# Autodesk Inventor assembly: Arcade
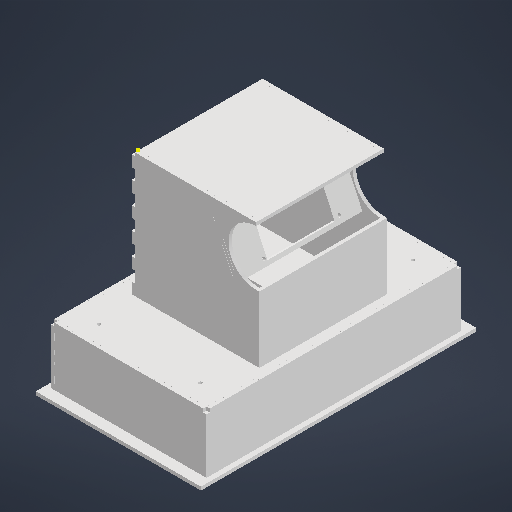
[picture p0: Inventor's stored thumbnail of the model, 512x512]
Saved by Autodesk Inventor 2026 (Build 300175000, 175)
## iProperties
Created: 2026-04-21
Part Number: Arcade
Document SubType Name: Assembly
Designer: juana
Author: juana
## Documents named in this file (9)
- C:\Users\juana\OneDrive\Documentos\GitHub\Digital_2\ModuloSTM32\ProyectoVideoJuegoF401RE\Arcade\Arcade.iam
- C:\Users\juana\OneDrive\Documentos\GitHub\Digital_2\ModuloSTM32\ProyectoVideoJuegoF401RE\Arcade\base.ipt
- C:\Users\juana\OneDrive\Documentos\GitHub\Digital_2\ModuloSTM32\ProyectoVideoJuegoF401RE\Arcade\AnchoBase.ipt
- C:\Users\juana\OneDrive\Documentos\GitHub\Digital_2\ModuloSTM32\ProyectoVideoJuegoF401RE\Arcade\paredBase.ipt
- C:\Users\juana\OneDrive\Documentos\GitHub\Digital_2\ModuloSTM32\ProyectoVideoJuegoF401RE\Arcade\ParedPantalla.ipt
- C:\Users\juana\OneDrive\Documentos\GitHub\Digital_2\ModuloSTM32\ProyectoVideoJuegoF401RE\Arcade\Techo.ipt
- C:\Users\juana\OneDrive\Documentos\GitHub\Digital_2\ModuloSTM32\ProyectoVideoJuegoF401RE\Arcade\portada.ipt
- C:\Users\juana\OneDrive\Documentos\GitHub\Digital_2\ModuloSTM32\ProyectoVideoJuegoF401RE\Arcade\pantallaSoport.ipt
- C:\Users\juana\OneDrive\Documentos\GitHub\Digital_2\ModuloSTM32\ProyectoVideoJuegoF401RE\Arcade\Techopantalla.ipt
## Components (11 placed, 8 different names)
1. base:1 — Mate:1, Mate:2, Flush:1, Mate:3, Mate:6, Flush:2, Mate:7, Mate:8
2. Techo:1 — Mate:9, Flush:3, Mate:10, Mate:11, Mate:12, Mate:13, Mate:14
3. portada:1 — Flush:4, Mate:14, Mate:15
4. pantallaSoport:1 — Flush:5, Mate:16, Mate:17
5. Techopantalla:1 — Mate:18, Flush:6, Mate:19
6. AnchoBase:1 — Flush:1, Mate:3, Mate:6, Flush:2
7. AnchoBase:3 — Flush:3, Mate:10
8. paredBase:1 — Mate:7, Mate:8, Mate:9
9. paredBase:2
10. ParedPantalla:1 — Mate:11, Mate:12, Mate:13, Flush:4, Flush:6, Mate:19
11. ParedPantalla:2 — Mate:15, Flush:5, Mate:16, Mate:17, Mate:18
## Component patterns: (2 elements, first: AnchoBase:1), (2 elements, first: paredBase:1), (2 elements, first: ParedPantalla:1)
## Relationships (23: Mate 17, Flush 6)
- Mate:1: base:1
- Mate:2: base:1
- Flush:1: base:1 ↔ AnchoBase:1
- Mate:3: base:1 ↔ AnchoBase:1
- Mate:6: base:1 ↔ AnchoBase:1
- Flush:2: base:1 ↔ AnchoBase:1
- Mate:7: base:1 ↔ paredBase:1
- Mate:8: base:1 ↔ paredBase:1
- Mate:9: Techo:1 ↔ paredBase:1
- Flush:3: Techo:1 ↔ AnchoBase:3
- Mate:10: Techo:1 ↔ AnchoBase:3
- Mate:11: Techo:1 ↔ ParedPantalla:1
- Mate:12: Techo:1 ↔ ParedPantalla:1
- Mate:13: Techo:1 ↔ ParedPantalla:1
- Flush:4: portada:1 ↔ ParedPantalla:1
- Mate:14: Techo:1 ↔ portada:1
- Mate:15: portada:1 ↔ ParedPantalla:2
- Flush:5: pantallaSoport:1 ↔ ParedPantalla:2
- Mate:16: pantallaSoport:1 ↔ ParedPantalla:2
- Mate:17: pantallaSoport:1 ↔ ParedPantalla:2
- Mate:18: Techopantalla:1 ↔ ParedPantalla:2
- Flush:6: Techopantalla:1 ↔ ParedPantalla:1
- Mate:19: Techopantalla:1 ↔ ParedPantalla:1
